# Autodesk Inventor assembly: Inverter Axle Combineinator
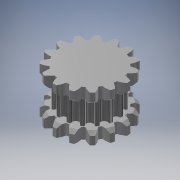
[picture p0: Inventor's stored thumbnail of the model, 180x180]
Saved by Autodesk Inventor 2019.4 (Build 234330000, 330)
## iProperties
Created: 2020-02-16
Part Number: Inverter Axle Combineinator
Document SubType Name: Assembly
Designer: admin
Author: admin
## Documents named in this file (3)
- C:\Users\admin\Desktop\FRC 2020 Engineering\GitHub\7738-2020\Robot V2\Storage System\3D printed Alternator\Inverter Axle Combineinator.iam
- C:\Users\admin\Desktop\FRC 2020 Engineering\GitHub\7738-2020\Robot V2\Storage System\3D printed Alternator\Inverter Axle.ipt
- C:\Users\admin\Desktop\FRC 2020 Engineering\GitHub\7738-2020\Robot V2\Storage System\3D printed Alternator\Inverter Axle Combineinator\Design Accelerator\Spur Gears1.iam
## Components (3 placed, 2 different names)
1. Inverter Axle:1 — Mate:1, Mate:2, Mate:3, Mate:4, Mate:5
2. Spur Gears:1 [sub-assembly] — Mate:1, Mate:2, Mate:3, Mate:6
3. Spur Gears:2 [sub-assembly] — Mate:4, Mate:5, Mate:6
## Relationships (6: Mate 6)
- Mate:1: Inverter Axle:1 ↔ Spur Gears:1
- Mate:2: Inverter Axle:1 ↔ Spur Gears:1
- Mate:3: Inverter Axle:1 ↔ Spur Gears:1
- Mate:4: Inverter Axle:1 ↔ Spur Gears:2
- Mate:5: Inverter Axle:1 ↔ Spur Gears:2
- Mate:6: Spur Gears:1 ↔ Spur Gears:2
